# Autodesk Inventor assembly: bottom_roller
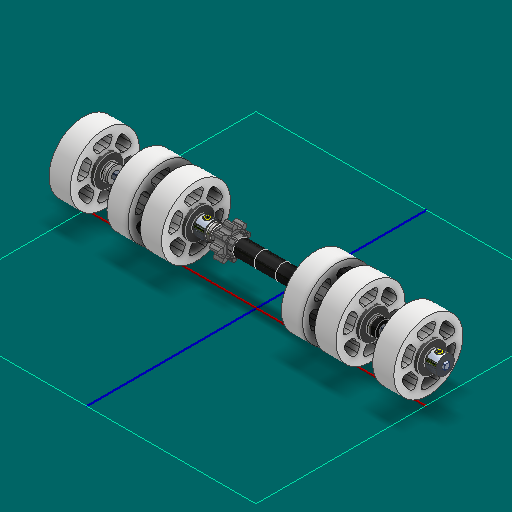
[picture p0: Inventor's stored thumbnail of the model, 512x512]
Saved by Autodesk Inventor 2025 (Build 290162000, 162)
## iProperties
Created: 2024-08-18
Part Number: bottom_roller
Document SubType Name: Assembly
Designer: averey
Author: averey
## Documents named in this file (18)
- C:\Users\avere\vex_robotics_high_stakes\hardware\cad\ATLAS\intake\first_stage\arm\bottom_roller.iam
- C:\Users\avere\vex_robotics_high_stakes\hardware\cad\_quick_assemblies\1.625_flex_wheel_w_versahex.iam
- C:\Users\avere\vex_robotics_high_stakes\hardware\cad\VEX-CAD-Inventor\Motion\Shaft LS\Shaft Collar ipts\Shaft Collar Set Screw.ipt
- C:\Users\avere\vex_robotics_high_stakes\hardware\cad\VEX-CAD-Inventor\Motion\Shaft LS\Shaft LS\Shaft LS 9.0.ipt
- C:\Users\avere\vex_robotics_high_stakes\hardware\cad\VEX-CAD-Inventor\Motion\Shaft LS\Shaft LS.ipt
- C:\Users\avere\vex_robotics_high_stakes\hardware\cad\VEX-CAD-Inventor\Motion\Spacers\Washer Teflon\TWasher .375 OD x .04000.ipt
- C:\Users\avere\vex_robotics_high_stakes\hardware\cad\VEX-CAD-Inventor\Motion\Spacers\Washer Teflon.ipt
- C:\Users\avere\vex_robotics_high_stakes\hardware\cad\VEX-CAD-Inventor\Motion\Spacers\Washer Teflon\TWasher .375 OD x .06250.ipt
- C:\Users\avere\vex_robotics_high_stakes\hardware\cad\VEX-CAD-Inventor\Motion\Spacers\Spacer Nylon .375 OD\NSpacer .375 OD x .500.ipt
- C:\Users\avere\vex_robotics_high_stakes\hardware\cad\VEX-CAD-Inventor\Motion\Spacers\Spacer Nylon .375 OD.ipt
- C:\Users\avere\vex_robotics_high_stakes\hardware\cad\VEX-CAD-Inventor\Motion\Spacers\Spacer Nylon .375 OD\NSpacer .375 OD x .375.ipt
- C:\Users\avere\vex_robotics_high_stakes\hardware\cad\VEX-CAD-Inventor\Motion\Spacers\Washer Steel\SWasher .375 OD x .015625.ipt
- C:\Users\avere\vex_robotics_high_stakes\hardware\cad\VEX-CAD-Inventor\Motion\Spacers\Washer Steel.ipt
- C:\Users\avere\vex_robotics_high_stakes\hardware\cad\VEX-CAD-Inventor\Motion\Spacers\Washer Steel\SWasher .375 OD x .031250.ipt
- C:\Users\avere\vex_robotics_high_stakes\hardware\cad\VEX-CAD-Inventor\Motion\Spacers\Spacer Nylon .375 OD\NSpacer .375 OD x .125.ipt
- C:\Users\avere\vex_robotics_high_stakes\hardware\cad\VEX-CAD-Inventor\Motion\Spacers\Washer Steel\SWasher .375 OD x .062500.ipt
- C:\Users\avere\vex_robotics_high_stakes\hardware\cad\VEX-CAD-Inventor\Motion\Sprockets\6P Sprocket\6P 8T Sprocket, Circle.iam
- C:\Users\avere\vex_robotics_high_stakes\hardware\cad\VEX-CAD-Inventor\Motion\Sprockets\6P Sprocket.iam
## Components (28 placed, 12 different names)
1. 1.625_flex_wheel_w_versahex:1 [sub-assembly] — Insert:1, Insert:7, Insert:8
2. 1.625_flex_wheel_w_versahex:2 [sub-assembly] — Insert:2, Insert:5
3. Shaft Collar Set Screw:1 — Insert:1, Insert:3, Mate:1
4. Shaft Collar Set Screw:2 — Insert:2, Flush:1, Mate:1
5. Shaft LS 9.0:1 — Insert:3, Flush:1
6. TWasher .375 OD x .04000:1 — Insert:4
7. TWasher .375 OD x .06250:2 — Insert:4, Insert:5
8. TWasher .375 OD x .04000:3 — Insert:6
9. TWasher .375 OD x .06250:4 — Insert:6, Insert:7
10. 1.625_flex_wheel_w_versahex:3 [sub-assembly] — Insert:8, Insert:11, Insert:21
11. 1.625_flex_wheel_w_versahex:4 [sub-assembly] — Insert:10, Insert:23
12. 1.625_flex_wheel_w_versahex:5 [sub-assembly] — Insert:10, Insert:13
13. 1.625_flex_wheel_w_versahex:6 [sub-assembly] — Insert:11, Insert:25
14. Shaft Collar Set Screw:3 — Insert:25
15. Shaft Collar Set Screw:4 — Insert:13, Insert:27
16. NSpacer .375 OD x .500:1 — Insert:16, Insert:17
17. NSpacer .375 OD x .500:2 — Insert:15, Insert:18, Insert:28
18. NSpacer .375 OD x .500:3 — Insert:17, Insert:18
19. NSpacer .375 OD x .375:4 — Insert:16
20. TWasher .375 OD x .04000:5 — Insert:14, Insert:15
21. SWasher .375 OD x .015625:1 — Insert:14, Insert:26
22. SWasher .375 OD x .031250:2 — Insert:20, Insert:21
23. NSpacer .375 OD x .125:5 — Insert:20
24. SWasher .375 OD x .031250:3
25. NSpacer .375 OD x .125:6 — Insert:23
26. SWasher .375 OD x .062500:4 — Insert:24, Insert:26
27. TWasher .375 OD x .04000:6 — Insert:24, Insert:27
28. 6P 8T Sprocket, Circle:1 [sub-assembly] — Insert:28
## Relationships (27: Insert 25, Flush 1, Mate 1)
- Insert:1: 1.625_flex_wheel_w_versahex:1 ↔ Shaft Collar Set Screw:1
- Insert:2: 1.625_flex_wheel_w_versahex:2 ↔ Shaft Collar Set Screw:2
- Insert:3 (-1.2019 mm): Shaft Collar Set Screw:1 ↔ Shaft LS 9.0:1
- Flush:1 (-1.2019 mm): Shaft Collar Set Screw:2 ↔ Shaft LS 9.0:1
- Mate:1: Shaft Collar Set Screw:1 ↔ Shaft Collar Set Screw:2
- Insert:4: TWasher .375 OD x .04000:1 ↔ TWasher .375 OD x .06250:2
- Insert:5: 1.625_flex_wheel_w_versahex:2 ↔ TWasher .375 OD x .06250:2
- Insert:6: TWasher .375 OD x .04000:3 ↔ TWasher .375 OD x .06250:4
- Insert:7: 1.625_flex_wheel_w_versahex:1 ↔ TWasher .375 OD x .06250:4
- Insert:8 (14.6162 mm): 1.625_flex_wheel_w_versahex:1 ↔ 1.625_flex_wheel_w_versahex:3
- Insert:10: 1.625_flex_wheel_w_versahex:4 ↔ 1.625_flex_wheel_w_versahex:5
- Insert:11: 1.625_flex_wheel_w_versahex:3 ↔ 1.625_flex_wheel_w_versahex:6
- Insert:13: 1.625_flex_wheel_w_versahex:5 ↔ Shaft Collar Set Screw:4
- Insert:14: TWasher .375 OD x .04000:5 ↔ SWasher .375 OD x .015625:1
- Insert:15: NSpacer .375 OD x .500:2 ↔ TWasher .375 OD x .04000:5
- Insert:16: NSpacer .375 OD x .500:1 ↔ NSpacer .375 OD x .375:4
- Insert:17: NSpacer .375 OD x .500:1 ↔ NSpacer .375 OD x .500:3
- Insert:18: NSpacer .375 OD x .500:2 ↔ NSpacer .375 OD x .500:3
- Insert:20: SWasher .375 OD x .031250:2 ↔ NSpacer .375 OD x .125:5
- Insert:21: 1.625_flex_wheel_w_versahex:3 ↔ SWasher .375 OD x .031250:2
- [Insert]: SWasher .375 OD x .031250:3 ↔ NSpacer .375 OD x .125:6
- Insert:23: 1.625_flex_wheel_w_versahex:4 ↔ NSpacer .375 OD x .125:6
- Insert:24: SWasher .375 OD x .062500:4 ↔ TWasher .375 OD x .04000:6
- Insert:25: 1.625_flex_wheel_w_versahex:6 ↔ Shaft Collar Set Screw:3
- Insert:26: SWasher .375 OD x .015625:1 ↔ SWasher .375 OD x .062500:4
- Insert:27: Shaft Collar Set Screw:4 ↔ TWasher .375 OD x .04000:6
- Insert:28: NSpacer .375 OD x .500:2 ↔ 6P 8T Sprocket, Circle:1
## Named parameters: d38_d36 = 0 mm
